# Autodesk Inventor assembly: Arrows
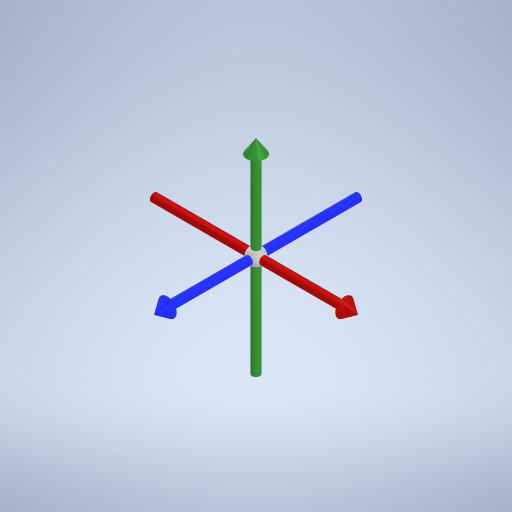
[picture p0: Inventor's stored thumbnail of the model, 512x512]
Saved by Autodesk Inventor 2023 (Build 270158000, 158)
## iProperties
Created: 2022-10-18
Part Number: Arrows
Document SubType Name: Assembly
Designer: benni
Author: benni
## Documents named in this file (3)
- C:\Users\benni\Documents\GitHub\IR_Assignment2\App Pictures\Arrows.iam
- C:\Users\benni\Documents\GitHub\IR_Assignment2\App Pictures\Center.ipt
- C:\Users\benni\Documents\GitHub\IR_Assignment2\App Pictures\Arrow.ipt
## Components (4 placed, 2 different names)
1. Center:1 — Mate:1, Mate:3
2. Arrow:1 — Mate:2, Mate:3
3. Arrow:2 — Mate:4, Mate:5
4. Arrow:3 — Mate:6, Mate:7
## Relationships (7: Mate 7)
- Mate:1: Center:1
- Mate:2: Arrow:1
- Mate:3 (-25 mm): Center:1 ↔ Arrow:1
- Mate:4: Arrow:2
- Mate:5 (-25 mm): Arrow:2
- Mate:6: Arrow:3
- Mate:7 (-25 mm): Arrow:3
